# Autodesk Inventor assembly: 110-01
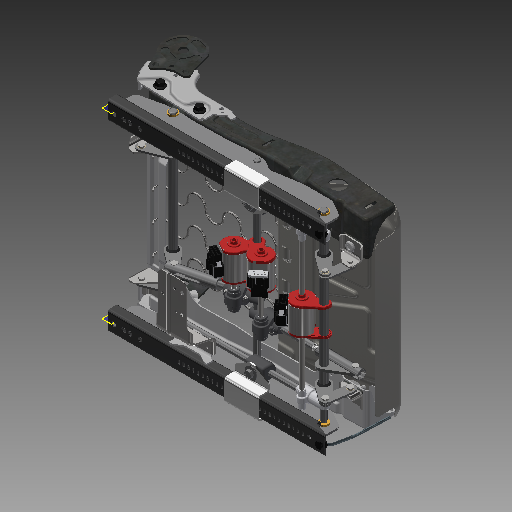
[picture p0: Inventor's stored thumbnail of the model, 512x512]
Saved by Autodesk Inventor 2019 (Build 230136000, 136)
## iProperties
Company: Autodesk Inc.
Created: 2007-12-24
Part Number: 110-01
Description: LOWER FULL ASSEMBLY
Document SubType Name: Assembly
Designer: Autodesk Inc.
Mass: 12502.3 g
Surface Area: 15972.1 cm^2
Volume: 1865.58 cm^3
Density: 6.70157 g/cm^3
Component Category: Lower Component
Author: Inventor
## Documents named in this file (21)
- C:\TEMP\Car Seat\Workspace\Lower Full Assembly_MIR.iam
- C:\TEMP\Car Seat\Workspace\Bottom Rail Assembly_MIR.iam
- C:\TEMP\Car Seat\Workspace\Bottom Guide Rail Assembly.iam
- C:\TEMP\Car Seat\Workspace\Pivot Plate.ipt
- C:\TEMP\Car Seat\Workspace\Pivot Link Weldment_MIR.iam
- C:\TEMP\Car Seat\Workspace\Ball Screw Sleeve.ipt
- C:\TEMP\Car Seat\Workspace\Pivot Pin A_MIR.ipt
- C:\TEMP\Car Seat\Workspace\Worm Gear Housing.ipt
- C:\TEMP\Car Seat\Workspace\Ball Screw Shaft B.ipt
- C:\TEMP\Car Seat\Workspace\Motor.iam
- C:\TEMP\Car Seat\Workspace\Pivot Rod.ipt
- C:\TEMP\Car Seat\Workspace\Back Support Plate L.ipt
- C:\TEMP\Car Seat\Workspace\Top Platform Mounting Bolt.ipt
- C:\TEMP\Car Seat\Workspace\Top Platform Mounting Nut.ipt
- C:\TEMP\Car Seat\Workspace\Back Support Plate R.ipt
- C:\TEMP\Car Seat\Workspace\Side Pivot Plate.ipt
- C:\TEMP\Car Seat\Workspace\Front Worm Drive Assembly_MIR.iam
- C:\TEMP\Car Seat\Workspace\Rear Worm Drive Assembly_MIR.iam
- C:\TEMP\Car Seat\Workspace\Front Link.ipt
- C:\TEMP\Car Seat\Workspace\Top Frame Assembly_MIR.iam
- C:\TEMP\Car Seat\Workspace\Front Pivot Links.iam
## Components (31 placed, 20 different names)
1. Bottom Rail Assembly_MIR:1 [sub-assembly] — Flush:9, Flush:8, Flush:7, Mate:2, Mate:5
2. Bottom Guide Rail Assembly:1 [sub-assembly] — Flush:12, Flush:11, Flush:10, Mate:11, Mate:3, Insert:18, Mate:41
3. Front Pivot Links:1 [sub-assembly] — Mate:15, Mate:1, Mate:6, Mate:10, Mate:31, Mate:32_1, Angle:1
4. Pivot Plate:1 — Mate:15, Mate:18, Mate:17, Angle:1
5. Pivot Link Weldment_MIR:1 [sub-assembly] — Mate:33_1, Mate:14, Mate:13, Insert:18
6. Top Frame Assembly_MIR:1 [sub-assembly] — Mate:33_1, Insert:21, Insert:12, Insert:22, Insert:25, Insert:19, Insert:20, Insert:19, Mate:33, Insert:20, Mate:34
7. Ball Screw Sleeve:1 — Mate:18, Mate:17, Tangent:1, Mate:21, Mate:16
8. Ball Screw Sleeve:2 — Mate:14, Mate:13, Mate:12
9. Pivot Pin A_MIR:1 — Tangent:1, Mate:21
10. Worm Gear Housing:1 — Mate:2, Mate:1, Insert:3
11. Worm Gear Housing:2 — Mate:6, Mate:5, Insert:18, Mate:7
12. Ball Screw Shaft B:1 — Insert:3
13. Ball Screw Shaft B:2 — Insert:18
14. Motor:1 [sub-assembly] — Mate:10, Mate:9
15. Pivot Rod:1 — Mate:9, Mate:8, Mate:7
16. Back Support Plate L:1 — Insert:19, Mate:33, Insert:23, Insert:24, Mate:35, Mate:36, Mate:37
17. Top Platform Mounting Bolt:1 — Insert:21
18. Top Platform Mounting Bolt:2 — Insert:22
19. Top Platform Mounting Nut:1 — Insert:21
20. Back Support Plate R:1 — Insert:20, Mate:34, Insert:21, Insert:22, Mate:38, Mate:39, Mate:40
21. Top Platform Mounting Nut:2 — Insert:12
22. Top Platform Mounting Bolt:3 — Insert:23
23. Top Platform Mounting Bolt:4 — Insert:24
24. Top Platform Mounting Nut:3 — Insert:22
25. Top Platform Mounting Nut:4 — Insert:25
26. Side Pivot Plate:1 — Mate:38, Mate:39, Mate:40
27. Side Pivot Plate:2 — Mate:35, Mate:36, Mate:37
28. Front Worm Drive Assembly_MIR:1 [sub-assembly] — Mate:11, Mate:16, Mate:3, Mate:30
29. Rear Worm Drive Assembly_MIR:1 [sub-assembly] — Mate:30, Mate:12, Mate:41
30. Front Link:1 — Insert:19, Mate:31
31. Front Link:2 — Insert:20, Mate:32_1
## Relationships (56: Mate 33, Insert 16, Flush 5, Tangent 1, Angle 1)
- Flush:9: Bottom Rail Assembly_MIR:1
- Flush:8: Bottom Rail Assembly_MIR:1
- Flush:7: Bottom Rail Assembly_MIR:1
- Flush:12 [Mate]: Bottom Guide Rail Assembly:1
- Flush:11 [Mate]: Bottom Guide Rail Assembly:1
- Flush:10: Bottom Guide Rail Assembly:1
- Mate:15: Front Pivot Links:1 ↔ Pivot Plate:1
- Mate:33_1: Pivot Link Weldment_MIR:1 ↔ Top Frame Assembly_MIR:1
- Mate:18: Pivot Plate:1 ↔ Ball Screw Sleeve:1
- Mate:17: Pivot Plate:1 ↔ Ball Screw Sleeve:1
- Mate:14: Pivot Link Weldment_MIR:1 ↔ Ball Screw Sleeve:2
- Mate:13: Pivot Link Weldment_MIR:1 ↔ Ball Screw Sleeve:2
- Tangent:1: Ball Screw Sleeve:1 ↔ Pivot Pin A_MIR:1
- Mate:21: Ball Screw Sleeve:1 ↔ Pivot Pin A_MIR:1
- Mate:2: Bottom Rail Assembly_MIR:1 ↔ Worm Gear Housing:1
- Mate:1: Front Pivot Links:1 ↔ Worm Gear Housing:1
- Mate:6: Front Pivot Links:1 ↔ Worm Gear Housing:2
- Mate:5: Bottom Rail Assembly_MIR:1 ↔ Worm Gear Housing:2
- Insert:3: Worm Gear Housing:1 ↔ Ball Screw Shaft B:1
- Insert:18: Worm Gear Housing:2 ↔ Ball Screw Shaft B:2
- Mate:10: Front Pivot Links:1 ↔ Motor:1
- Mate:9: Motor:1 ↔ Pivot Rod:1
- Mate:8 [Flush]: Pivot Rod:1
- Mate:7: Worm Gear Housing:2 ↔ Pivot Rod:1
- Insert:21: Top Frame Assembly_MIR:1 ↔ Top Platform Mounting Nut:1
- Insert:12: Top Frame Assembly_MIR:1 ↔ Top Platform Mounting Nut:2
- Insert:22: Top Frame Assembly_MIR:1 ↔ Top Platform Mounting Nut:3
- Insert:25: Top Frame Assembly_MIR:1 ↔ Top Platform Mounting Nut:4
- Mate:11: Bottom Guide Rail Assembly:1 ↔ Front Worm Drive Assembly_MIR:1
- Mate:16: Ball Screw Sleeve:1 ↔ Front Worm Drive Assembly_MIR:1
- Mate:3: Bottom Guide Rail Assembly:1 ↔ Front Worm Drive Assembly_MIR:1
- Mate:30: Front Worm Drive Assembly_MIR:1 ↔ Rear Worm Drive Assembly_MIR:1
- Mate:12: Ball Screw Sleeve:2 ↔ Rear Worm Drive Assembly_MIR:1
- Insert:19: Top Frame Assembly_MIR:1 ↔ Front Link:1
- Mate:31: Front Pivot Links:1 ↔ Front Link:1
- Insert:20: Top Frame Assembly_MIR:1 ↔ Front Link:2
- Mate:32_1: Front Pivot Links:1 ↔ Front Link:2
- [Insert]: Bottom Guide Rail Assembly:1 ↔ Front Pivot Links:1
- Insert:18: Bottom Guide Rail Assembly:1 ↔ Pivot Link Weldment_MIR:1
- [Mate] (0.5 mm): Front Pivot Links:1 ↔ Front Link:1
- Insert:19: Top Frame Assembly_MIR:1 ↔ Back Support Plate L:1
- Mate:33: Top Frame Assembly_MIR:1 ↔ Back Support Plate L:1
- Insert:20: Top Frame Assembly_MIR:1 ↔ Back Support Plate R:1
- Mate:34: Top Frame Assembly_MIR:1 ↔ Back Support Plate R:1
- Insert:21: Top Platform Mounting Bolt:1 ↔ Back Support Plate R:1
- Insert:22: Top Platform Mounting Bolt:2 ↔ Back Support Plate R:1
- Insert:23: Back Support Plate L:1 ↔ Top Platform Mounting Bolt:3
- Insert:24: Back Support Plate L:1 ↔ Top Platform Mounting Bolt:4
- Mate:35: Back Support Plate L:1 ↔ Side Pivot Plate:2
- Mate:36: Back Support Plate L:1 ↔ Side Pivot Plate:2
- Mate:37: Back Support Plate L:1 ↔ Side Pivot Plate:2
- Mate:38: Back Support Plate R:1 ↔ Side Pivot Plate:1
- Mate:39: Back Support Plate R:1 ↔ Side Pivot Plate:1
- Mate:40: Back Support Plate R:1 ↔ Side Pivot Plate:1
- Angle:1 (-100 deg): Front Pivot Links:1 ↔ Pivot Plate:1
- Mate:41: Bottom Guide Rail Assembly:1 ↔ Rear Worm Drive Assembly_MIR:1
